# Autodesk Inventor assembly: Toolhead_PCB
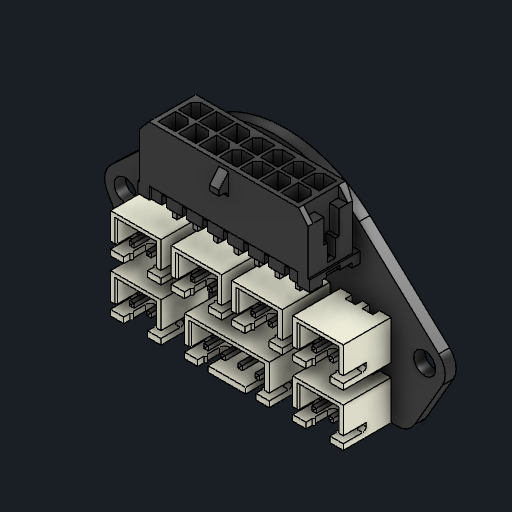
[picture p0: Inventor's stored thumbnail of the model, 512x512]
Saved by Autodesk Inventor 2026.1 (Build 301233020, 233B)
## iProperties
Company: A Company
Created: 2021-06-02
Part Number: Toolhead_PCB
Description: KiCad electronic assembly
Document SubType Name: Assembly
Designer: Joshua Eah
Authority: Unknown
Sending System: KiCad to STEP converter
Preprocessor: Open CASCADE STEP processor 6.9
Title: Toolhead_PCB.step
Author: An Author
## Documents named in this file (5)
- C:\Users\JoshuaEah\Documents\GitHub\Voron-0\CAD\Master Assembly\Toolhead\Subassemblies\Toolhead_PCB.iam
- C:\Users\JoshuaEah\Documents\GitHub\Voron-0\CAD\Master Assembly\Electronics\Parts\Toolhead PCB.ipt
- C:\Users\JoshuaEah\Documents\GitHub\Voron-0\CAD\Master Assembly\Electronics\Parts\JST XH 4 Pin Female.ipt
- C:\Users\JoshuaEah\Documents\GitHub\Voron-0\CAD\Master Assembly\Electronics\Parts\JST XH 2 Pin Female.ipt
- C:\Users\JoshuaEah\Documents\GitHub\Voron-0\CAD\Master Assembly\Electronics\Parts\Molex 14 Pin Female 90 Degree.ipt
## Components (9 placed, 4 different names)
1. JST-XH 2 Pin Female:1
2. JST-XH 2 Pin Female:2
3. JST-XH 2 Pin Female:3
4. JST-XH 2 Pin Female:4
5. JST-XH 2 Pin Female:5
6. JST-XH 2 Pin Female:6
7. JST-XH 4 Pin Female:1
8. Molex 14 Pin
9. Toolhead PCB
## Named parameters: Finish3_Area = 23.7764
note: some values were not read from the file. Shown as the stored number, unit unknown: "Finish3_Area".
